# Autodesk Inventor assembly: gusset
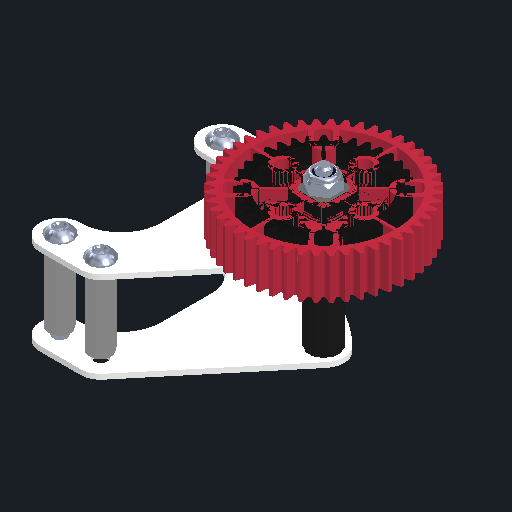
[picture p0: Inventor's stored thumbnail of the model, 512x512]
Saved by Autodesk Inventor 2025 (Build 290162000, 162)
## iProperties
Created: 2024-08-21
Part Number: gusset
Document SubType Name: Assembly
Designer: averey
Author: averey
## Documents named in this file (7)
- D:\vex_robotics_high_stakes\hardware\cad\bots\ENIGMA\chassis\drivetrain\drivebay\gusset.iam
- D:\vex_robotics_high_stakes\hardware\cad\bots\ENIGMA\chassis\drivetrain\drivebay\custom_parts\gusset.ipt
- C:\Users\avere\vex_robotics_high_stakes\hardware\cad\VEX-CAD-Inventor\Structure\Standoff.ipt
- D:\vex_robotics_high_stakes\hardware\cad\VEX-CAD-Inventor\Structure\Standoff\Standoff .875.ipt
- D:\vex_robotics_high_stakes\hardware\cad\VEX-CAD-Inventor\Structure\Hardware\Screw Shoulder Robosource\SScrew Shoulder Smooth .290 x .09.ipt
- C:\Users\avere\vex_robotics_high_stakes\hardware\cad\VEX-CAD-Inventor\Structure\Hardware\Screw Shoulder Robosource.ipt
- D:\vex_robotics_high_stakes\hardware\cad\bots\ENIGMA\chassis\drivetrain\drivebay\wall_glides.iam
## Components (13 placed, 4 different names)
1. gusset:1 — Insert:1, Mate:1, Insert:3, Insert:4, Insert:6
2. gusset:2 — Insert:1, Mate:1, Insert:5
3. wall_glides:1 [sub-assembly] — Insert:6
4. SScrew Shoulder Smooth .290 x .09:5 — Insert:5
5. SScrew Shoulder Smooth .290 x .09:6
6. Standoff .875:2 — Insert:3
7. Standoff .875:3
8. Standoff .875:4
9. Standoff .875:5
10. SScrew Shoulder Smooth .290 x .09:1 — Insert:4
11. SScrew Shoulder Smooth .290 x .09:2
12. SScrew Shoulder Smooth .290 x .09:3
13. SScrew Shoulder Smooth .290 x .09:4
## Component patterns: (2 elements, first: SScrew Shoulder Smooth .290 x .09:5), Standoffs (4 elements), Top Screws (4 elements)
## Relationships (6: Insert 5, Mate 1)
- Insert:1 (25.4 mm): gusset:1 ↔ gusset:2
- Mate:1: gusset:1 ↔ gusset:2
- Insert:3 (1.5875 mm): gusset:1 ↔ Standoff .875:2
- Insert:4: gusset:1 ↔ SScrew Shoulder Smooth .290 x .09:1
- Insert:5: gusset:2 ↔ SScrew Shoulder Smooth .290 x .09:5
- Insert:6: gusset:1 ↔ wall_glides:1
